# Autodesk Inventor assembly: leg_ass_1_MIR
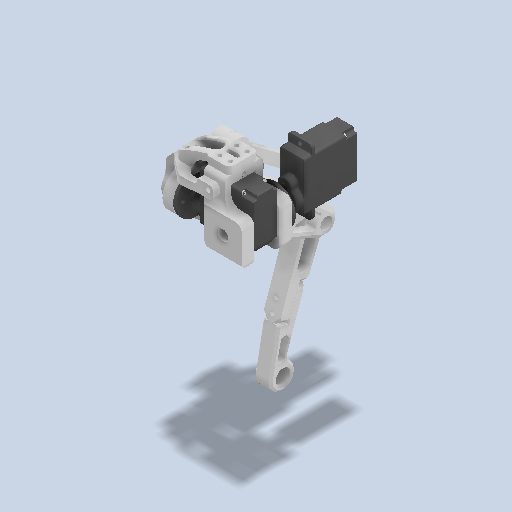
[picture p0: Inventor's stored thumbnail of the model, 512x512]
Saved by Autodesk Inventor 2022.1 (Build 261234020, 234B)
## iProperties
Created: 2019-09-26
Part Number: leg_ass_1_MIR
Document SubType Name: Assembly
Designer: kee
Mass: 55.2074 g
Surface Area: 287.547 cm^2
Volume: 46.1036 cm^3
Density: 1.19746 g/cm^3
Author: kee
## Documents named in this file (11)
- C:\Users\logic\_workspace\Quadruped_bai_servo\hardware\inventor\quadruped_bai_servo_assembly\leg_ass_1_MIR.iam
- C:\Users\logic\_workspace\Quadruped_bai_servo\hardware\inventor\quadruped_bai_servo_assembly\Emax ES08A_MIR.ipt
- C:\Users\logic\_workspace\Quadruped_bai_servo\hardware\inventor\quadruped_bai_servo_assembly\leg_1_MIR.ipt
- C:\Users\logic\_workspace\Quadruped_bai_servo\hardware\inventor\quadruped_bai_servo_assembly\leg_2_MIR.ipt
- C:\Users\logic\_workspace\Quadruped_bai_servo\hardware\inventor\quadruped_bai_servo_assembly\leg_1_2_MIR.ipt
- C:\Users\logic\_workspace\Quadruped_bai_servo\hardware\inventor\quadruped_bai_servo_assembly\leg_link_1_MIR.ipt
- C:\Users\logic\_workspace\Quadruped_bai_servo\hardware\inventor\quadruped_bai_servo_assembly\leg_link-1_MIR.ipt
- C:\Users\logic\_workspace\Quadruped_bai_servo\hardware\inventor\quadruped_bai_servo_assembly\leg_tip_MIR.ipt
- C:\Users\logic\_workspace\Quadruped_bai_servo\hardware\inventor\quadruped_bai_servo_assembly\servo_holder_1_MIR1.ipt
- C:\Users\logic\_workspace\Quadruped_bai_servo\hardware\inventor\quadruped_bai_servo_assembly\hip_joint_holder_1_MIR.ipt
- C:\Users\logic\_workspace\Quadruped_bai_servo\hardware\inventor\quadruped_bai_servo_assembly\hip_holder_2_MIR.ipt
## Components (12 placed, 10 different names)
1. Emax ES08A_MIR:1 — Insert:9, Insert:10, Mate:1
2. leg_1_MIR:1 — Rotational:1, Insert:9, Insert:10, Rotational:4, Insert:11, Insert:12
3. Emax ES08A_MIR:2 — Insert:5, Insert:6
4. leg_2_MIR:1 — Rotational:4, Insert:13, Insert:14, Rotational:5
5. leg_1_2_MIR:1 — Insert:11, Insert:12
6. leg_link_1_MIR:1 — Rotational:3, Mate:1
7. leg_link-1_MIR:1 — Rotational:3, Rotational:5
8. leg_tip_MIR:1 — Insert:13, Insert:14
9. servo_holder_1_MIR1:1 — Insert:1, Insert:4, Insert:5, Insert:6, Insert:7, Insert:8, Flush:1
10. Emax ES08A_MIR:3 — Insert:7, Insert:8
11. hip_joint_holder_1_MIR:1 — Rotational:1, Insert:3, Insert:4
12. hip_holder_2_MIR:1 — Insert:1, Insert:3, Flush:2
## Relationships (20: Insert 13, RevoluteJoint 4, Flush 2, Mate 1)
- Insert:1: servo_holder_1_MIR1:1 ↔ hip_holder_2_MIR:1
- Rotational:1 [RevoluteJoint]: leg_1_MIR:1 ↔ hip_joint_holder_1_MIR:1
- Insert:3: hip_joint_holder_1_MIR:1 ↔ hip_holder_2_MIR:1
- Insert:4: servo_holder_1_MIR1:1 ↔ hip_joint_holder_1_MIR:1
- Insert:5: Emax ES08A_MIR:2 ↔ servo_holder_1_MIR1:1
- Insert:6: Emax ES08A_MIR:2 ↔ servo_holder_1_MIR1:1
- Insert:7: servo_holder_1_MIR1:1 ↔ Emax ES08A_MIR:3
- Insert:8: servo_holder_1_MIR1:1 ↔ Emax ES08A_MIR:3
- Insert:9: Emax ES08A_MIR:1 ↔ leg_1_MIR:1
- Insert:10: Emax ES08A_MIR:1 ↔ leg_1_MIR:1
- Rotational:3 [RevoluteJoint]: leg_link_1_MIR:1 ↔ leg_link-1_MIR:1
- Rotational:4 [RevoluteJoint]: leg_1_MIR:1 ↔ leg_2_MIR:1
- Insert:11: leg_1_MIR:1 ↔ leg_1_2_MIR:1
- Insert:12: leg_1_MIR:1 ↔ leg_1_2_MIR:1
- Insert:13: leg_2_MIR:1 ↔ leg_tip_MIR:1
- Insert:14: leg_2_MIR:1 ↔ leg_tip_MIR:1
- Rotational:5 [RevoluteJoint]: leg_2_MIR:1 ↔ leg_link-1_MIR:1
- Mate:1: Emax ES08A_MIR:1 ↔ leg_link_1_MIR:1
- Flush:1: servo_holder_1_MIR1:1
- Flush:2: hip_holder_2_MIR:1
